# Autodesk Inventor assembly: servo_metallic_600TVL
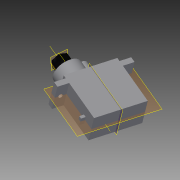
[picture p0: Inventor's stored thumbnail of the model, 180x180]
Saved by Autodesk Inventor 2015 SP1 (Build 190203100, 203)
## iProperties
Created: 2015-07-09
Part Number: servo_metallic_600TVL
Document SubType Name: Assembly
Designer: Alexandre Cherpillod
Author: Alexandre Cherpillod
## Documents named in this file (3)
- D:\_windows\_github_doc\MAVRIC\Mechanics\myCopter_CAD\servo_FatShark_180MG.iam
- D:\_windows\_github_doc\MAVRIC\Mechanics\myCopter_CAD\servo_FatShark_180MG.ipt
- D:\_windows\_github_doc\MAVRIC\Mechanics\myCopter_CAD\shaft_nut_for_FatShark_180MG.ipt
## Components (2 placed, 2 different names)
1. servo_FatShark_180MG:1 — Mate:1, Flush:1
2. shaft_nut_for_FatShark_180MG:1 — Mate:1, Flush:1
## Relationships (2: Mate 1, Flush 1)
- Mate:1: servo_FatShark_180MG:1 ↔ shaft_nut_for_FatShark_180MG:1
- Flush:1 (-11.5 mm): servo_FatShark_180MG:1 ↔ shaft_nut_for_FatShark_180MG:1
